# Autodesk Inventor assembly: Assembly1
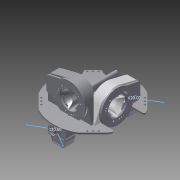
[picture p0: Inventor's stored thumbnail of the model, 180x180]
Saved by Autodesk Inventor 2011 (Build 150239000, 239)
## iProperties
Created: 2011-03-18
Part Number: Assembly1
Document SubType Name: Assembly
Designer: casey
Author: casey
## Documents named in this file (7)
- C:\Users\M. Woods III\Desktop\design\Mechanical Drawings\assembly.iam
- C:\Users\M. Woods III\Desktop\design\Mechanical Drawings\Rocket\deck.ipt
- C:\Users\M. Woods III\Desktop\design\Mechanical Drawings\launcher_1.iam
- C:\Users\M. Woods III\Desktop\design\Mechanical Drawings\camera.iam
- C:\Users\M. Woods III\Desktop\design\Mechanical Drawings\pusher_1.iam
- C:\Users\M. Woods III\Desktop\design\Mechanical Drawings\launcher_2.iam
- C:\Users\M. Woods III\Desktop\design\Mechanical Drawings\pusher_2.iam
## Components (7 placed, 6 different names)
1. deck:1 — Mate:9, Mate:12, Mate:13, Mate:14, Mate:15, Mate:16, Mate:19, Mate:22, Mate:29, Mate:32, Mate:33
2. camera:1 [sub-assembly] — Mate:9
3. camera:3 [sub-assembly] — Mate:12
4. launcher_1:1 [sub-assembly] — Mate:13, Mate:14, Mate:15, Mate:16, Mate:34
5. pusher_1:1 [sub-assembly] — Mate:19, Mate:31, Mate:34
6. launcher_2:1 [sub-assembly] — Mate:22, Angle:1, Mate:32, Mate:33, Mate:35
7. pusher_2:1 [sub-assembly] — Mate:29, Flush:1, Mate:31, Mate:35
## Relationships (16: Mate 14, Flush 1, Angle 1)
- Mate:9: deck:1 ↔ camera:1
- Mate:12: deck:1 ↔ camera:3
- Mate:13: deck:1 ↔ launcher_1:1
- Mate:14: deck:1 ↔ launcher_1:1
- Mate:15: deck:1 ↔ launcher_1:1
- Mate:16: deck:1 ↔ launcher_1:1
- Mate:19: deck:1 ↔ pusher_1:1
- Mate:22: deck:1 ↔ launcher_2:1
- Mate:29: deck:1 ↔ pusher_2:1
- Flush:1: pusher_2:1
- Angle:1 (0 deg): launcher_2:1
- Mate:31: pusher_1:1 ↔ pusher_2:1
- Mate:32: deck:1 ↔ launcher_2:1
- Mate:33: deck:1 ↔ launcher_2:1
- Mate:34: launcher_1:1 ↔ pusher_1:1
- Mate:35: launcher_2:1 ↔ pusher_2:1
